# Autodesk Inventor assembly: _WandAssembly
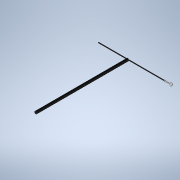
[picture p0: Inventor's stored thumbnail of the model, 180x180]
Saved by Autodesk Inventor 2022 (Build 260153000, 153)
## iProperties
Created: 2022-06-22
Part Number: _WandAssembly
Document SubType Name: Assembly
Designer: tecware
Author: tecware
## Documents named in this file (4)
- C:\Users\tecware\Documents\git\calibrationKit\calibrationKit_v2\wand\_WandAssembly.iam
- C:\Users\tecware\Documents\git\calibrationKit\calibrationKit_v2\wand\components_wand\horizontalRod.ipt
- C:\Users\tecware\Documents\git\calibrationKit\calibrationKit_v2\wand\components_wand\PVC_conduit.ipt
- C:\Users\tecware\Documents\git\calibrationKit\calibrationKit_v2\wand\components_wand\markerWithRodEnd_new1.ipt
## Components (4 placed, 3 different names)
1. horizontalRod:1 — Mate:2, Mate:3
2. PVC_conduit:1
3. markerWithRodEnd_new1:1 — Mate:1, Flush:1, Mate:3, Mate:4
4. markerWithRodEnd_new1:2 — Mate:1, Flush:1, Mate:2, Mate:4
## Relationships (5: Mate 4, Flush 1)
- Mate:1: markerWithRodEnd_new1:1 ↔ markerWithRodEnd_new1:2
- Flush:1: markerWithRodEnd_new1:1 ↔ markerWithRodEnd_new1:2
- Mate:2: horizontalRod:1 ↔ markerWithRodEnd_new1:2
- Mate:3: horizontalRod:1 ↔ markerWithRodEnd_new1:1
- Mate:4: markerWithRodEnd_new1:1 ↔ markerWithRodEnd_new1:2
